# Autodesk Inventor assembly: PistaoEquipado2
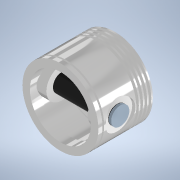
[picture p0: Inventor's stored thumbnail of the model, 180x180]
Saved by Autodesk Inventor 2021 (Build 250183000, 183)
## iProperties
Created: 2021-07-24
Part Number: PistaoEquipado2
Document SubType Name: Assembly
Designer: Giovanni
Author: Giovanni
## Documents named in this file (4)
- C:\Users\irineu\Documents\Inventor\MotorRadial7\PistaoEquipado2.iam
- C:\Users\irineu\Documents\Inventor\MotorRadial7\Pistão1.ipt
- C:\Users\irineu\Documents\Inventor\MotorRadial7\Pino_Pistão1.ipt
- C:\Users\irineu\Documents\Inventor\MotorRadial7\Plug_Pistão1.ipt
## Components (4 placed, 3 different names)
1. Pistão1:1 — Coincidente:1
2. Pino_Pistão1:1 — Coincidente:1, Coincidente:2, Inserir:1, Inserir:2
3. Plug_Pistão1:1 — Inserir:1
4. Plug_Pistão1:2 — Inserir:2
## Relationships (4: Mate 2, Insert 2)
- Coincidente:1 [Mate]: Pistão1:1 ↔ Pino_Pistão1:1
- Coincidente:2 [Mate]: Pino_Pistão1:1
- Inserir:1: Pino_Pistão1:1 ↔ Plug_Pistão1:1
- Inserir:2: Pino_Pistão1:1 ↔ Plug_Pistão1:2
